# Autodesk Inventor assembly: Balboa32U4_Body
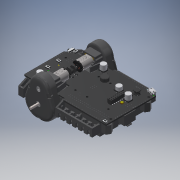
[picture p0: Inventor's stored thumbnail of the model, 180x180]
Saved by Autodesk Inventor 2018 (Build 220112000, 112)
## iProperties
Created: 2017-12-26
Part Number: Balboa32U4_Body
Material: 一般
Description: STEP AP214
Document SubType Name: Assembly
Designer: ku_sk
Mass: 147.6 g
Surface Area: 802.962 cm^2
Volume: 93.8476 cm^3
Density: 1.57276 g/cm^3
Sending System: SolidWorks 2016
Preprocessor: SwSTEP 2.0
Title: balboa-balancing-robot-kit.step
Revision Number: ANY
## Documents named in this file (4)
- D:\Inventor\Balboa32U4-CAD\parts\Body\Balboa32U4_Body.iam
- D:\Inventor\Balboa32U4-CAD\parts\Body\parts\chassis.ipt
- D:\Inventor\Balboa32U4-CAD\parts\Body\parts\battery-cover.ipt
- D:\Inventor\Balboa32U4-CAD\parts\Body\parts\circuit.ipt
## Components (3 placed, 3 different names)
1. chassis_1 — フラッシュ:1, フラッシュ:2, メイト:1, メイト:2, 角度:1, メイト:3, メイト:8, メイト:9, メイト:10
2. battery-cover_2 — メイト:8, メイト:9, メイト:10
3. circuit — フラッシュ:1, フラッシュ:2, メイト:1
## Relationships (9: Mate 6, Flush 2, Angle 1)
- フラッシュ:1 [Flush]: chassis_1 ↔ circuit
- フラッシュ:2 [Flush] (-19.86 mm): chassis_1 ↔ circuit
- メイト:1 [Mate]: chassis_1 ↔ circuit
- メイト:2 [Mate]: chassis_1
- 角度:1 [Angle] (0 deg): chassis_1
- メイト:3 [Mate]: chassis_1
- メイト:8 [Mate]: chassis_1 ↔ battery-cover_2
- メイト:9 [Mate]: chassis_1 ↔ battery-cover_2
- メイト:10 [Mate] (0.15 mm): chassis_1 ↔ battery-cover_2
